# Autodesk Inventor assembly: 6 Perf Plaction Tread 500 Hex
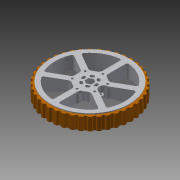
[picture p0: Inventor's stored thumbnail of the model, 180x180]
Saved by Autodesk Inventor 2013 (Build 170138000, 138)
## iProperties
Created: 2013-02-07
Part Number: 6 Perf Plaction Tread 500 Hex
Document SubType Name: Assembly
Designer: Moses
Author: Moses
## Documents named in this file (3)
- C:\Users\Moses\Documents\GitHub\frc2013CAD\Drivetrain\6 Perf ThruTread 500 Hex\6 Perf Plaction Tread 500 Hex.iam
- C:\Users\Moses\Documents\GitHub\frc2013CAD\Drivetrain\6 Perf ThruTread 500 Hex\6 Perf ThruTread 500 Hex.ipt
- C:\Users\Moses\Documents\GitHub\frc2013CAD\Drivetrain\6 Perf ThruTread 500 Hex\6plactiontread.ipt
## Components (2 placed, 2 different names)
1. 6 Perf ThruTread 500 Hex:1 — Mate:1, Mate:2
2. 6plactiontread:1 — Mate:1, Mate:2
## Relationships (2: Mate 2)
- Mate:1: 6 Perf ThruTread 500 Hex:1 ↔ 6plactiontread:1
- Mate:2 (1.524 mm): 6 Perf ThruTread 500 Hex:1 ↔ 6plactiontread:1
